# Autodesk Inventor assembly: PWTR-0147
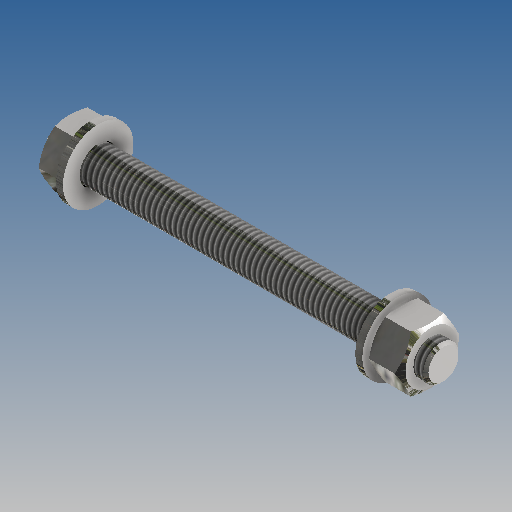
[picture p0: Inventor's stored thumbnail of the model, 512x512]
Saved by Autodesk Inventor 2021.1 (Build 251245000, 245)
## iProperties
Created: 2020-09-02
Part Number: PWTR-0147
Document SubType Name: Assembly
Designer: alid
Description: Arm Fastener
Author: alid
Revision Number: A
## Documents named in this file (4)
- C:\Vault Workspace\Design Data\Projects\PRJ0095\PWTR-CTO\PWTR-0147.iam
- C:\Vault Workspace\Design Data\Projects\PRJ0095\PWTR-CTO\PWTR-0148.ipt
- C:\Vault Workspace\Design Data\Projects\PRJ0095\PWTR-CTO\PWTR-0149.ipt
- C:\Vault Workspace\Design Data\Projects\PRJ0095\PWTR-CTO\PWTR-0150.ipt
## Components (4 placed, 3 different names)
1. PWTR-0148:1
2. PWTR-0150:1
3. PWTR-0149:1 — Insert:3
4. PWTR-0149:2 — Insert:3
## Relationships (3: Insert 3)
- [Insert]: PWTR-0148:1 ↔ PWTR-0149:1
- [Insert]: PWTR-0150:1 ↔ PWTR-0149:2
- Insert:3 (83 mm): PWTR-0149:1 ↔ PWTR-0149:2
